# Autodesk Inventor assembly: hinge
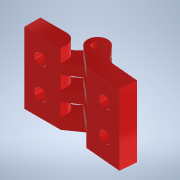
[picture p0: Inventor's stored thumbnail of the model, 180x180]
Saved by Autodesk Inventor 2022 (Build 260153000, 153)
## iProperties
Created: 2022-08-02
Part Number: hinge
Document SubType Name: Assembly
Designer: thoma
Author: thoma
## Documents named in this file (2)
- C:\Users\thoma\OneDrive\Documents\CREATION\Serre\hinge.iam
- C:\Users\thoma\OneDrive\Documents\CREATION\Serre\halfhinge.ipt
## Components (2 placed, 1 different names)
1. halfhinge:1 — Mate:1, Mate:2
2. halfhinge:2 — Mate:1, Mate:2
## Relationships (2: Mate 2)
- Mate:1: halfhinge:1 ↔ halfhinge:2
- Mate:2 (0.6 mm): halfhinge:1 ↔ halfhinge:2
